# Autodesk Inventor assembly: Lift assembly left
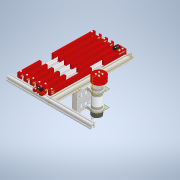
[picture p0: Inventor's stored thumbnail of the model, 180x180]
Saved by Autodesk Inventor 2020 (Build 240168000, 168)
## iProperties
Created: 2019-11-17
Part Number: Lift assembly left
Document SubType Name: Assembly
Designer: ball
Author: ball
## Documents named in this file (18)
- D:\FTC8863\2019 Robot\Delivery\Lift assembly left.iam
- D:\FTC8863\Actobotics\605 parts\605630.ipt
- D:\FTC8863\StepLibraries\Nuts\2-56 NYLON-INSERT LOCKNUT.ipt
- D:\FTC8863\StepLibraries\Screws\M3 x 25 HEX HEAD CAP SCREW.ipt
- D:\FTC8863\2019 Robot\Delivery\Limit switch trigger spacer.ipt
- D:\FTC8863\Actobotics\565 parts\xrail_3.5in.ipt
- D:\FTC8863\Actobotics\555 parts\555116 assembly.ipt
- D:\FTC8863\2019 Robot\Generic Parts\limit switch mount to xrail.ipt
- D:\FTC8863\StepLibraries\Screws\2-56x.5_18-8 SS PAN HEAD PHILLIPS MACHINE SCREW.ipt
- D:\FTC8863\StepLibraries\Screws\6-32x.375_18-8 SS TRUSS HEAD PHILLIPS MACHINE SCREW.ipt
- D:\FTC8863\2019 Robot\Delivery\Limit switch top + mount left.iam
- D:\FTC8863\2019 Robot\Delivery\Coupler lift long left bracket + pulleys.iam
- D:\FTC8863\2019 Robot\Delivery\SAR330  x 5 + couplers left.iam
- D:\FTC8863\2019 Robot\Delivery\Coupler lift short left + pulleys.iam
- D:\FTC8863\Actobotics\585 parts\585721.ipt
- D:\FTC8863\2019 Robot\Delivery\spool double 2 in diameter.iam
- D:\FTC8863\Andymark\am-2964a Neverest Classic 40.ipt
- D:\FTC8863\StepLibraries\Screws\565050.ipt
## Components (22 placed, 17 different names)
1. SAR330  x 5 + couplers left:1 [sub-assembly] — Mate:5, Flush:7, Mate:18, Mate:19, Mate:33, Mate:34, Mate:35, Mate:36, Flush:16, Mate:40, Flush:21, Flush:34, Flush:35, Mate:68, Mate:72, Mate:73, Mate:74, Mate:113, Flush:42, Flush:43
2. 605630:2 — Mate:5, Flush:7, Flush:33, Mate:61, Mate:63, Mate:64, Mate:65
3. M3 x 25 HEX HEAD CAP SCREW:1 — Mate:18, Mate:19, Mate:25, Mate:26
4. Limit switch trigger spacer:1 — Mate:25, Mate:26
5. M3 x 25 HEX HEAD CAP SCREW:2 — Mate:33, Mate:109
6. M3 x 25 HEX HEAD CAP SCREW:3 — Mate:34, Mate:110
7. Coupler lift short left + pulleys:1 [sub-assembly] — Mate:35, Mate:36, Flush:16
8. 565050:1
9. xrail_3.5in:1 — Mate:40, Flush:21, Flush:39, Mate:112, Flush:41
10. 555116 assembly:1 — Mate:118, Mate:119, Mate:120, Mate:121
11. 555116 assembly:2 — Mate:115, Mate:116, Mate:117, Mate:119, Mate:120
12. limit switch mount to xrail:1 — Flush:33, Mate:61, Mate:62, Angle:1, Mate:66, Mate:67
13. 2-56 NYLON-INSERT LOCKNUT:4 — Mate:62, Mate:63, Angle:1
14. 2-56x.5_18-8 SS PAN HEAD PHILLIPS MACHINE SCREW:1 — Mate:64, Mate:65
15. 6-32x.375_18-8 SS TRUSS HEAD PHILLIPS MACHINE SCREW:1 — Mate:66, Mate:67
16. Limit switch top + mount left:1 [sub-assembly] — Flush:34, Flush:35, Mate:68, Mate:109, Mate:110
17. Coupler lift long left bracket + pulleys:1 [sub-assembly] — Mate:72, Mate:73, Mate:74
18. spool double 2 in diameter:1 [sub-assembly] — Mate:106, Mate:107, Flush:42
19. am-2964a Neverest Classic 40:1 — Mate:106, Mate:107, Mate:121
20. xrail_3.5in:3 — Mate:114, Flush:41, Flush:43
21. 585721:3 — Flush:39, Mate:112, Flush:40, Mate:114, Mate:116, Mate:117
22. 585721:4 — Flush:40, Mate:113, Mate:115, Mate:118
## Relationships (55: Mate 38, Flush 16, Angle 1)
- Mate:5 (1.27 mm): SAR330  x 5 + couplers left:1 ↔ 605630:2
- Flush:7: SAR330  x 5 + couplers left:1 ↔ 605630:2
- Mate:18: SAR330  x 5 + couplers left:1 ↔ M3 x 25 HEX HEAD CAP SCREW:1
- Mate:19 (6 mm): SAR330  x 5 + couplers left:1 ↔ M3 x 25 HEX HEAD CAP SCREW:1
- Mate:25: M3 x 25 HEX HEAD CAP SCREW:1 ↔ Limit switch trigger spacer:1
- Mate:26: M3 x 25 HEX HEAD CAP SCREW:1 ↔ Limit switch trigger spacer:1
- Mate:33: SAR330  x 5 + couplers left:1 ↔ M3 x 25 HEX HEAD CAP SCREW:2
- Mate:34: SAR330  x 5 + couplers left:1 ↔ M3 x 25 HEX HEAD CAP SCREW:3
- Mate:35: SAR330  x 5 + couplers left:1 ↔ Coupler lift short left + pulleys:1
- Mate:36: SAR330  x 5 + couplers left:1 ↔ Coupler lift short left + pulleys:1
- Flush:16: SAR330  x 5 + couplers left:1 ↔ Coupler lift short left + pulleys:1
- [Flush]: Coupler lift short left + pulleys:1 ↔ 565050:1
- [Mate]: Coupler lift short left + pulleys:1 ↔ 565050:1
- Mate:40: SAR330  x 5 + couplers left:1 ↔ xrail_3.5in:1
- Flush:21: SAR330  x 5 + couplers left:1 ↔ xrail_3.5in:1
- [Mate]: 565050:1 ↔ limit switch mount to xrail:1
- [Flush]: 565050:1 ↔ limit switch mount to xrail:1
- Flush:33: 605630:2 ↔ limit switch mount to xrail:1
- Mate:61: 605630:2 ↔ limit switch mount to xrail:1
- Mate:62: limit switch mount to xrail:1 ↔ 2-56 NYLON-INSERT LOCKNUT:4
- Mate:63: 605630:2 ↔ 2-56 NYLON-INSERT LOCKNUT:4
- Angle:1 (0 deg): limit switch mount to xrail:1 ↔ 2-56 NYLON-INSERT LOCKNUT:4
- Mate:64: 605630:2 ↔ 2-56x.5_18-8 SS PAN HEAD PHILLIPS MACHINE SCREW:1
- Mate:65: 605630:2 ↔ 2-56x.5_18-8 SS PAN HEAD PHILLIPS MACHINE SCREW:1
- Mate:66: limit switch mount to xrail:1 ↔ 6-32x.375_18-8 SS TRUSS HEAD PHILLIPS MACHINE SCREW:1
- Mate:67: limit switch mount to xrail:1 ↔ 6-32x.375_18-8 SS TRUSS HEAD PHILLIPS MACHINE SCREW:1
- Flush:34: SAR330  x 5 + couplers left:1 ↔ Limit switch top + mount left:1
- Flush:35 (2.54 mm): SAR330  x 5 + couplers left:1 ↔ Limit switch top + mount left:1
- Mate:68: SAR330  x 5 + couplers left:1 ↔ Limit switch top + mount left:1
- Mate:72: SAR330  x 5 + couplers left:1 ↔ Coupler lift long left bracket + pulleys:1
- Mate:73: SAR330  x 5 + couplers left:1 ↔ Coupler lift long left bracket + pulleys:1
- Mate:74: SAR330  x 5 + couplers left:1 ↔ Coupler lift long left bracket + pulleys:1
- Mate:106: spool double 2 in diameter:1 ↔ am-2964a Neverest Classic 40:1
- Mate:107: spool double 2 in diameter:1 ↔ am-2964a Neverest Classic 40:1
- Mate:109: M3 x 25 HEX HEAD CAP SCREW:2 ↔ Limit switch top + mount left:1
- Mate:110: M3 x 25 HEX HEAD CAP SCREW:3 ↔ Limit switch top + mount left:1
- [Mate]: 585721:3 ↔ 585721:4
- [Flush]: 585721:3 ↔ 585721:4
- [Flush]: xrail_3.5in:3 ↔ 585721:3
- Flush:39: xrail_3.5in:1 ↔ 585721:3
- Mate:112: xrail_3.5in:1 ↔ 585721:3
- Flush:40: 585721:3 ↔ 585721:4
- Mate:113: SAR330  x 5 + couplers left:1 ↔ 585721:4
- Mate:114: xrail_3.5in:3 ↔ 585721:3
- Flush:41: xrail_3.5in:1 ↔ xrail_3.5in:3
- Mate:115: 555116 assembly:2 ↔ 585721:4
- Mate:116: 555116 assembly:2 ↔ 585721:3
- Mate:117: 555116 assembly:2 ↔ 585721:3
- Mate:118: 555116 assembly:1 ↔ 585721:4
- Mate:119: 555116 assembly:1 ↔ 555116 assembly:2
- Mate:120 (55.5244 mm): 555116 assembly:1 ↔ 555116 assembly:2
- Mate:121: 555116 assembly:1 ↔ am-2964a Neverest Classic 40:1
- Flush:42 (-8.0264 mm): SAR330  x 5 + couplers left:1 ↔ spool double 2 in diameter:1
- Flush:43 (120.65 mm): SAR330  x 5 + couplers left:1 ↔ xrail_3.5in:3
- [Flush] (-25.2476 mm): Coupler lift short left + pulleys:1 ↔ 565050:1
## Named parameters: d204_d100 = 0 mm
